# Autodesk Inventor assembly: Montagem
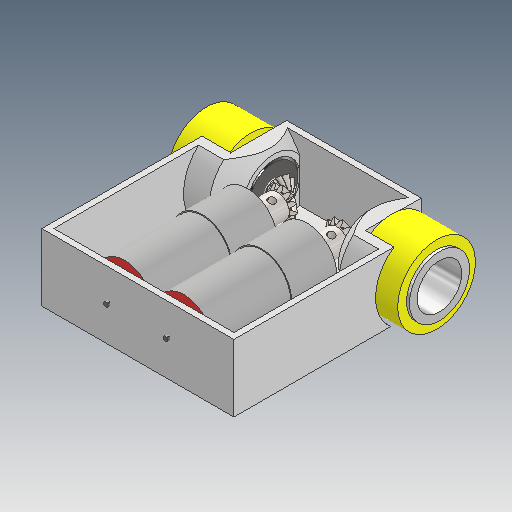
[picture p0: Inventor's stored thumbnail of the model, 512x512]
Saved by Autodesk Inventor 2026.1 (Build 301233020, 233B)
## iProperties
Created: 2025-11-09
Part Number: Montagem
Document SubType Name: Assembly
Designer: Emmanuel Ribeiro
Author: Emmanuel Ribeiro
## Documents named in this file (9)
- C:\Users\sonel\Desktop\Robô Rebeca\Montagem.iam
- C:\Users\sonel\Desktop\Robô Rebeca\arruela.ipt
- C:\Users\sonel\Desktop\Robô Rebeca\Bucha.ipt
- C:\Users\sonel\Desktop\Robô Rebeca\Engrenagem conica 1.ipt
- C:\Users\sonel\Desktop\Robô Rebeca\Engrenagem conica 2.ipt
- C:\Users\sonel\Desktop\Robô Rebeca\Motor.ipt
- C:\Users\sonel\Desktop\Robô Rebeca\Roda.ipt
- C:\Users\sonel\Desktop\Robô Rebeca\rolamento.ipt
- C:\Users\sonel\Desktop\Robô Rebeca\Base.ipt
## Components (15 placed, 8 different names)
1. arruela:1 — Coincidente:7, Coincidente:8
2. Bucha:1 — Coincidente:3, Coincidente:4, Coincidente:5, Coincidente:6
3. Engrenagem conica 1:1 — Coincidente:11, Coincidente:12
4. Engrenagem conica 2:1 — Coincidente:1, Coincidente:4, Coincidente:14
5. Motor:1 — Coincidente:11, Coincidente:12, Tangente:1, Tangente:3, Alinhado:1
6. Roda:1 — Coincidente:5, Coincidente:6, Coincidente:7, Coincidente:8, Coincidente:13
7. rolamento:1 — Coincidente:1, Coincidente:3, Coincidente:14, Coincidente:15
8. Base:1 — Coincidente:13, Tangente:1, Coincidente:15, Tangente:2, Coincidente:26, Coincidente:27
9. arruela:2
10. Bucha:2
11. Engrenagem conica 1:2
12. Engrenagem conica 2:2
13. Motor:2 — Tangente:2, Tangente:3, Alinhado:1
14. Roda:2
15. rolamento:2 — Coincidente:26, Coincidente:27
## Relationships (28: Mate 24, Tangent 3, Flush 1)
- Coincidente:1 [Mate]: Engrenagem conica 2:1 ↔ rolamento:1
- Coincidente:3 [Mate]: Bucha:1 ↔ rolamento:1
- Coincidente:4 [Mate]: Bucha:1 ↔ Engrenagem conica 2:1
- Coincidente:5 [Mate]: Bucha:1 ↔ Roda:1
- Coincidente:6 [Mate]: Bucha:1 ↔ Roda:1
- Coincidente:7 [Mate]: arruela:1 ↔ Roda:1
- Coincidente:8 [Mate]: arruela:1 ↔ Roda:1
- Coincidente:11 [Mate]: Engrenagem conica 1:1 ↔ Motor:1
- Coincidente:12 [Mate]: Engrenagem conica 1:1 ↔ Motor:1
- Coincidente:13 [Mate]: Roda:1 ↔ Base:1
- Tangente:1: Motor:1 ↔ Base:1
- Coincidente:14 [Mate]: Engrenagem conica 2:1 ↔ rolamento:1
- Coincidente:15 [Mate]: rolamento:1 ↔ Base:1
- [Mate]: Engrenagem conica 2:2 ↔ rolamento:2
- [Mate]: Bucha:2 ↔ rolamento:2
- [Mate]: Bucha:2 ↔ Engrenagem conica 2:2
- [Mate]: Bucha:2 ↔ Roda:2
- [Mate]: Bucha:2 ↔ Roda:2
- [Mate]: arruela:2 ↔ Roda:2
- [Mate]: arruela:2 ↔ Roda:2
- [Mate]: Engrenagem conica 1:2 ↔ Motor:2
- [Mate]: Engrenagem conica 1:2 ↔ Motor:2
- [Mate]: Engrenagem conica 2:2 ↔ rolamento:2
- Tangente:2: Base:1 ↔ Motor:2
- Tangente:3: Motor:1 ↔ Motor:2
- Alinhado:1 [Flush]: Motor:1 ↔ Motor:2
- Coincidente:26 [Mate]: Base:1 ↔ rolamento:2
- Coincidente:27 [Mate]: Base:1 ↔ rolamento:2
## Named parameters: d17_d0 = 0 mm, d18_d2 = 0 mm, d19_d3 = 0 mm, d20_d4 = 0 mm, d21_d5 = 0 mm, d22_d7 = 0 mm, d23_d8 = 0 mm, d24_d11 = 0 mm, d25_d12 = 0 mm, d26_d15 = 0 mm
